# Autodesk Inventor assembly: Robot
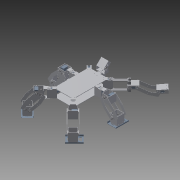
[picture p0: Inventor's stored thumbnail of the model, 180x180]
Saved by Autodesk Inventor 2013 (Build 170138000, 138)
## iProperties
Created: 2014-05-11
Part Number: Robot
Document SubType Name: Assembly
Designer: andou
Author: andou
## Documents named in this file (7)
- C:\Users\andou\Documents\Inventor\RoboticsProject\project_4\Robot\Robot.iam
- C:\Users\andou\Documents\Inventor\RoboticsProject\project_4\Robot\Body\Main Plate.ipt
- C:\Users\andou\Documents\Inventor\RoboticsProject\project_4\Robot\Leg\Left_Leg\Left Leg.iam
- C:\Users\andou\Documents\Inventor\RoboticsProject\project_4\Robot\Leg\Right_Leg\Right Leg.iam
- C:\Users\andou\Documents\Inventor\RoboticsProject\project_4\Robot\Head\Head.iam
- C:\Users\andou\Documents\Inventor\RoboticsProject\project_4\Robot\Arm\Left_Arm.iam
- C:\Users\andou\Documents\Inventor\RoboticsProject\project_4\Robot\Arm\Right_Arm.iam
## Components (9 placed, 6 different names)
1. Main Plate:1 — 挿入:1, 挿入:2, 挿入:3, 挿入:4, 挿入:5, 挿入:6, 挿入:7, 挿入:8, 挿入:9, 挿入:10, 挿入:13, 挿入:14, 挿入:15, 挿入:16, 挿入:17, 挿入:18, 挿入:19, 挿入:20, 挿入:21, 挿入:22, 挿入:33, 挿入:34, 挿入:35, 挿入:36
2. Main Plate:2 — 挿入:11, 挿入:12, 挿入:23, 挿入:24, 挿入:25, 挿入:26, 挿入:27, 挿入:28, 挿入:29, 挿入:30, 挿入:31, 挿入:32
3. Left Leg:1 [sub-assembly] — 挿入:2, 挿入:3, 挿入:12, 挿入:13, 挿入:19, 挿入:31, 挿入:32
4. Left Leg:2 [sub-assembly] — 挿入:1, 挿入:4, 挿入:14, 挿入:20, 挿入:29, 挿入:30
5. Right Leg:1 [sub-assembly] — 挿入:8, 挿入:9, 挿入:16, 挿入:17, 挿入:25, 挿入:26
6. Right Leg:2 [sub-assembly] — 挿入:7, 挿入:10, 挿入:11, 挿入:15, 挿入:18, 挿入:27, 挿入:28
7. Head:1 [sub-assembly] — 挿入:5, 挿入:6, 挿入:21, 挿入:22, 挿入:23, 挿入:24
8. Left_Arm:1 [sub-assembly] — 挿入:33, 挿入:34
9. Right_Arm:1 [sub-assembly] — 挿入:35, 挿入:36
## Relationships (36: Insert 36)
- 挿入:1 [Insert]: Main Plate:1 ↔ Left Leg:2
- 挿入:2 [Insert]: Main Plate:1 ↔ Left Leg:1
- 挿入:3 [Insert]: Main Plate:1 ↔ Left Leg:1
- 挿入:4 [Insert]: Main Plate:1 ↔ Left Leg:2
- 挿入:5 [Insert]: Main Plate:1 ↔ Head:1
- 挿入:6 [Insert]: Main Plate:1 ↔ Head:1
- 挿入:7 [Insert]: Main Plate:1 ↔ Right Leg:2
- 挿入:8 [Insert]: Main Plate:1 ↔ Right Leg:1
- 挿入:9 [Insert]: Main Plate:1 ↔ Right Leg:1
- 挿入:10 [Insert]: Main Plate:1 ↔ Right Leg:2
- 挿入:11 [Insert]: Main Plate:2 ↔ Right Leg:2
- 挿入:12 [Insert]: Main Plate:2 ↔ Left Leg:1
- 挿入:13 [Insert]: Main Plate:1 ↔ Left Leg:1
- 挿入:14 [Insert]: Main Plate:1 ↔ Left Leg:2
- 挿入:15 [Insert]: Main Plate:1 ↔ Right Leg:2
- 挿入:16 [Insert]: Main Plate:1 ↔ Right Leg:1
- 挿入:17 [Insert]: Main Plate:1 ↔ Right Leg:1
- 挿入:18 [Insert]: Main Plate:1 ↔ Right Leg:2
- 挿入:19 [Insert]: Main Plate:1 ↔ Left Leg:1
- 挿入:20 [Insert]: Main Plate:1 ↔ Left Leg:2
- 挿入:21 [Insert]: Main Plate:1 ↔ Head:1
- 挿入:22 [Insert]: Main Plate:1 ↔ Head:1
- 挿入:23 [Insert]: Main Plate:2 ↔ Head:1
- 挿入:24 [Insert]: Main Plate:2 ↔ Head:1
- 挿入:25 [Insert]: Main Plate:2 ↔ Right Leg:1
- 挿入:26 [Insert]: Main Plate:2 ↔ Right Leg:1
- 挿入:27 [Insert]: Main Plate:2 ↔ Right Leg:2
- 挿入:28 [Insert]: Main Plate:2 ↔ Right Leg:2
- 挿入:29 [Insert]: Main Plate:2 ↔ Left Leg:2
- 挿入:30 [Insert]: Main Plate:2 ↔ Left Leg:2
- 挿入:31 [Insert]: Main Plate:2 ↔ Left Leg:1
- 挿入:32 [Insert]: Main Plate:2 ↔ Left Leg:1
- 挿入:33 [Insert]: Main Plate:1 ↔ Left_Arm:1
- 挿入:34 [Insert]: Main Plate:1 ↔ Left_Arm:1
- 挿入:35 [Insert]: Main Plate:1 ↔ Right_Arm:1
- 挿入:36 [Insert]: Main Plate:1 ↔ Right_Arm:1
